# Autodesk Inventor assembly: ASY GBK центральная стенка
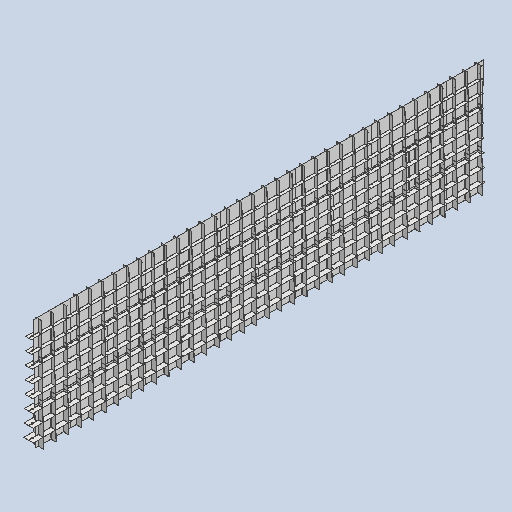
[picture p0: Inventor's stored thumbnail of the model, 512x512]
Saved by Autodesk Inventor 2026.2 (Build 302298000, 298)
## iProperties
Created: 2026-05-28
Part Number: ASY GBK центральная стенка
Document SubType Name: Assembly
Designer: pokla
Stock Number: 3000
Author: pokla
## Documents named in this file (10)
- C:\Users\admin\Documents\Inventor\GBK-Gubkinskiy\ASY GBK центральная стенка.iam
- C:\Users\admin\Documents\Inventor\GBK-Gubkinskiy\ASY GBK 3110 central wall shield 1.iam
- C:\Users\admin\Documents\Inventor\GBK-Gubkinskiy\ASY GBK 3120 central wall shield 2.iam
- C:\Users\admin\Documents\Inventor\GBK-Gubkinskiy\ASY GBK 3210 central wall shield 4.iam
- C:\Users\admin\Documents\Inventor\GBK-Gubkinskiy\ASY GBK 3220 central wall shield 5.iam
- C:\Users\admin\Documents\Inventor\GBK-Gubkinskiy\ASY GBK 3310 central wall shield 7.iam
- C:\Users\admin\Documents\Inventor\GBK-Gubkinskiy\ASY GBK 3320 central wall shield 8.iam
- C:\Users\admin\Documents\Inventor\GBK-Gubkinskiy\ASY GBK 3330 central wall shield 9.iam
- C:\Users\admin\Documents\Inventor\GBK-Gubkinskiy\ASY GBK 3230 central wall shield 6.iam
- C:\Users\admin\Documents\Inventor\GBK-Gubkinskiy\ASY GBK 3130 central wall shield 3.iam
## Components (20 placed, 12 different names)
1. ASY GBK 3110 central wall shield 1.iam:1 [sub-assembly] — Mate:1, Rigid:1, Mate:4, Mate:5, Flush:1, Mate:6
2. ASY GBK 3120 central wall shield 2.iam:1 [sub-assembly] — Rigid:1, Rigid:6
3. ASY GBK 3210 central wall shield 4.iam:1 [sub-assembly] — Rigid:3, Mate:5, Flush:1, Mate:6, Mate:7, Flush:2, Mate:8
4. ASY GBK 3220 central wall shield 5.iam:1 [sub-assembly] — Rigid:3, Rigid:11
5. ASY GBK 3310 central wall shield 7.iam:1 [sub-assembly] — Rigid:5, Mate:7, Flush:2, Mate:8
6. ASY GBK 3320 central wall shield 8.iam:1 [sub-assembly] — Rigid:5, Rigid:15
7. ASY GBK 3330 central wall shield 9.iam:1 [sub-assembly] — Rigid:19
8. ASY GBK 3230 central wall shield 6.iam:1 [sub-assembly] — Rigid:14
9. ASY GBK 3130 central wall shield 3.iam:1 [sub-assembly] — Rigid:10
10. ASY GBK 3120 central wall shield 2:2 [sub-assembly] — Rigid:6, Rigid:7
11. ASY GBK 3120 central wall shield 2:3 [sub-assembly] — Rigid:7, Rigid:8
12. ASY GBK 3120 central wall shield 2:4 [sub-assembly] — Rigid:8, Rigid:9
13. ASY GBK 3120 central wall shield 2:5 [sub-assembly] — Rigid:9, Rigid:10
14. ASY GBK 3220 central wall shield 4:2 [sub-assembly] — Rigid:11, Rigid:12
15. ASY GBK 3220 central wall shield 4:3 [sub-assembly] — Rigid:12, Rigid:13
16. ASY GBK 3220 central wall shield 4:4 [sub-assembly] — Rigid:13, Rigid:14
17. ASY GBK 3320 central wall shield 8:2 [sub-assembly] — Rigid:15, Rigid:16
18. ASY GBK 3320 central wall shield 8:3 [sub-assembly] — Rigid:16, Rigid:17
19. ASY GBK 3320 central wall shield 8:4 [sub-assembly] — Rigid:17, Rigid:18
20. ASY GBK 3320 central wall shield 8:5 [sub-assembly] — Rigid:18, Rigid:19
## Relationships (25: WeldJoint 17, Mate 6, Flush 2)
- Mate:1: ASY GBK 3110 central wall shield 1.iam:1
- Rigid:1 [WeldJoint] (1 mm): ASY GBK 3110 central wall shield 1.iam:1 ↔ ASY GBK 3120 central wall shield 2.iam:1
- Mate:4: ASY GBK 3110 central wall shield 1.iam:1
- Rigid:3 [WeldJoint] (1 mm): ASY GBK 3210 central wall shield 4.iam:1 ↔ ASY GBK 3220 central wall shield 5.iam:1
- Rigid:5 [WeldJoint] (1 mm): ASY GBK 3310 central wall shield 7.iam:1 ↔ ASY GBK 3320 central wall shield 8.iam:1
- Rigid:6 [WeldJoint] (1 mm): ASY GBK 3120 central wall shield 2.iam:1 ↔ ASY GBK 3120 central wall shield 2:2
- Rigid:7 [WeldJoint] (1 mm): ASY GBK 3120 central wall shield 2:2 ↔ ASY GBK 3120 central wall shield 2:3
- Rigid:8 [WeldJoint] (1 mm): ASY GBK 3120 central wall shield 2:3 ↔ ASY GBK 3120 central wall shield 2:4
- Rigid:9 [WeldJoint] (1 mm): ASY GBK 3120 central wall shield 2:4 ↔ ASY GBK 3120 central wall shield 2:5
- Rigid:10 [WeldJoint] (1 mm): ASY GBK 3130 central wall shield 3.iam:1 ↔ ASY GBK 3120 central wall shield 2:5
- Rigid:11 [WeldJoint] (1 mm): ASY GBK 3220 central wall shield 5.iam:1 ↔ ASY GBK 3220 central wall shield 4:2
- Rigid:12 [WeldJoint] (1 mm): ASY GBK 3220 central wall shield 4:2 ↔ ASY GBK 3220 central wall shield 4:3
- Rigid:13 [WeldJoint] (1 mm): ASY GBK 3220 central wall shield 4:3 ↔ ASY GBK 3220 central wall shield 4:4
- Rigid:14 [WeldJoint] (1 mm): ASY GBK 3230 central wall shield 6.iam:1 ↔ ASY GBK 3220 central wall shield 4:4
- Rigid:15 [WeldJoint] (1 mm): ASY GBK 3320 central wall shield 8.iam:1 ↔ ASY GBK 3320 central wall shield 8:2
- Rigid:16 [WeldJoint] (1 mm): ASY GBK 3320 central wall shield 8:2 ↔ ASY GBK 3320 central wall shield 8:3
- Rigid:17 [WeldJoint] (1 mm): ASY GBK 3320 central wall shield 8:3 ↔ ASY GBK 3320 central wall shield 8:4
- Rigid:18 [WeldJoint] (1 mm): ASY GBK 3320 central wall shield 8:4 ↔ ASY GBK 3320 central wall shield 8:5
- Rigid:19 [WeldJoint] (1 mm): ASY GBK 3330 central wall shield 9.iam:1 ↔ ASY GBK 3320 central wall shield 8:5
- Mate:5 (1 mm): ASY GBK 3110 central wall shield 1.iam:1 ↔ ASY GBK 3210 central wall shield 4.iam:1
- Flush:1: ASY GBK 3110 central wall shield 1.iam:1 ↔ ASY GBK 3210 central wall shield 4.iam:1
- Mate:6 (1 mm): ASY GBK 3110 central wall shield 1.iam:1 ↔ ASY GBK 3210 central wall shield 4.iam:1
- Mate:7 (1 mm): ASY GBK 3210 central wall shield 4.iam:1 ↔ ASY GBK 3310 central wall shield 7.iam:1
- Flush:2: ASY GBK 3210 central wall shield 4.iam:1 ↔ ASY GBK 3310 central wall shield 7.iam:1
- Mate:8 (1 mm): ASY GBK 3210 central wall shield 4.iam:1 ↔ ASY GBK 3310 central wall shield 7.iam:1
